# Autodesk Inventor assembly: ASY Beshkino main
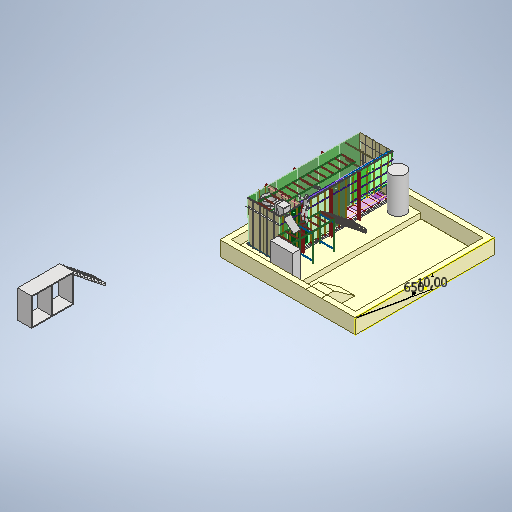
[picture p0: Inventor's stored thumbnail of the model, 512x512]
Saved by Autodesk Inventor 2025 (Build 290162010, 162A)
## iProperties
Created: 2024-08-27
Part Number: ASY Beshkino main
Document SubType Name: Assembly
Designer: DELL
Author: DELL
## Documents named in this file (13)
- C:\Users\DELL\YandexDisk-badmisterfox\домашниий пк\Inventor\BSH_Beshkino_bio_tank\ASY Beshkino main.iam
- C:\Users\DELL\YandexDisk-badmisterfox\домашниий пк\Inventor\BSH_Beshkino_bio_tank\BSH 0 foudation.ipt
- C:\Users\DELL\YandexDisk-badmisterfox\домашниий пк\Inventor\BSH_Beshkino_bio_tank\ASY Beshkino_bio_tank.iam
- C:\Users\DELL\YandexDisk-badmisterfox\домашниий пк\Inventor\BSH_Beshkino_bio_tank\ASY Trommel.iam
- C:\Users\DELL\YandexDisk-badmisterfox\домашниий пк\Inventor\BSH_Beshkino_bio_tank\3d party\RXm3 assieme dimensionale mag2018.ipt
- C:\Users\DELL\YandexDisk-badmisterfox\домашниий пк\Inventor\BSH_Beshkino_bio_tank\3d party\motor-reductor NMRV040\motor-reductor NMRV040.iam
- C:\Users\DELL\YandexDisk-badmisterfox\домашниий пк\Inventor\BSH_Beshkino_bio_tank\BSH 01 foam filter.ipt
- C:\Users\DELL\YandexDisk-badmisterfox\домашниий пк\Inventor\BSH_Beshkino_bio_tank\BSH 01 bag.ipt
- C:\Users\DELL\YandexDisk-badmisterfox\домашниий пк\Inventor\BSH_Beshkino_bio_tank\BSH 03 upstairs.ipt
- C:\Users\DELL\YandexDisk-badmisterfox\домашниий пк\Inventor\BSH_Beshkino_bio_tank\Конструкция.iam
- C:\Users\DELL\YandexDisk-badmisterfox\домашниий пк\Inventor\BSH_Beshkino_bio_tank\лестница\Перегородка\ASY NDM 11.030 перегородка рама 2 горизонт.iam
- C:\Users\DELL\YandexDisk-badmisterfox\домашниий пк\Inventor\BSH_Beshkino_bio_tank\ISO 657_15 - SB 140x15 - 3000.ipt
- C:\Users\DELL\YandexDisk-badmisterfox\домашниий пк\Inventor\BSH_Beshkino_bio_tank\лестница\dummi\human 01\ч ASY human dummy 01.iam
## Components (19 placed, 12 different names)
1. BSH 0 foudation:1 — Mate:1, Mate:2, Mate:3, Mate:4, Flush:2, Flush:3, Flush:4, Mate:7
2. ASY Beshkino_bio_tank:1 [sub-assembly] — Mate:2, Mate:3, Mate:4, Flush:1, Mate:5, Mate:6, Mate:8, Mate:10, Flush:7, Mate:14
3. ASY Trommel:1 [sub-assembly] — Flush:1
4. RXm3 assieme dimensionale mag2018:1 — Mate:5
5. RXm3 assieme dimensionale mag2018:2 — Mate:6
6. motor-reductor NMRV040:1 [sub-assembly]
7. BSH 01 foam filter:1 — Flush:2
8. BSH 01 bag:1 — Flush:3
9. BSH 03 upstairs:1 — Flush:4
10. Конструкция:1 [sub-assembly] — Mate:7, Mate:8, Mate:13
11. ASY NDM 11.030 перегородка рама 2 горизонт:1 [sub-assembly] — Flush:5, Flush:6, Mate:9, Mate:10
12. ASY NDM 11.030 перегородка рама 2 горизонт:2 [sub-assembly] — Flush:5, Flush:6, Mate:9
13. ч ASY human dummy 01:1 [sub-assembly] — Mate:13
14. ISO 657_15 - SB 140x15 - 3000:1 — Flush:7, Mate:14
15. ISO 657_15 - SB 140x15 - 3000:2
16. ISO 657_15 - SB 140x15 - 3000:3
17. ISO 657_15 - SB 140x15 - 3000:4
18. ISO 657_15 - SB 140x15 - 3000:5
19. ISO 657_15 - SB 140x15 - 3000:6
## Component patterns: (6 elements, first: ISO 657_15 - SB 140x15 - 3000:1)
## Relationships (19: Mate 12, Flush 7)
- Mate:1: BSH 0 foudation:1
- Mate:2: BSH 0 foudation:1 ↔ ASY Beshkino_bio_tank:1
- Mate:3 (100 mm): BSH 0 foudation:1 ↔ ASY Beshkino_bio_tank:1
- Mate:4 (200 mm): BSH 0 foudation:1 ↔ ASY Beshkino_bio_tank:1
- Flush:1: ASY Beshkino_bio_tank:1 ↔ ASY Trommel:1
- Mate:5: ASY Beshkino_bio_tank:1 ↔ RXm3 assieme dimensionale mag2018:1
- Mate:6: ASY Beshkino_bio_tank:1 ↔ RXm3 assieme dimensionale mag2018:2
- Flush:2: BSH 0 foudation:1 ↔ BSH 01 foam filter:1
- Flush:3: BSH 0 foudation:1 ↔ BSH 01 bag:1
- Flush:4: BSH 0 foudation:1 ↔ BSH 03 upstairs:1
- Mate:7: BSH 0 foudation:1 ↔ Конструкция:1
- Mate:8 (140 mm): ASY Beshkino_bio_tank:1 ↔ Конструкция:1
- Flush:5: ASY NDM 11.030 перегородка рама 2 горизонт:1 ↔ ASY NDM 11.030 перегородка рама 2 горизонт:2
- Flush:6: ASY NDM 11.030 перегородка рама 2 горизонт:1 ↔ ASY NDM 11.030 перегородка рама 2 горизонт:2
- Mate:9: ASY NDM 11.030 перегородка рама 2 горизонт:1 ↔ ASY NDM 11.030 перегородка рама 2 горизонт:2
- Mate:10: ASY Beshkino_bio_tank:1 ↔ ASY NDM 11.030 перегородка рама 2 горизонт:1
- Mate:13: Конструкция:1 ↔ ч ASY human dummy 01:1
- Flush:7 (1500 mm): ASY Beshkino_bio_tank:1 ↔ ISO 657_15 - SB 140x15 - 3000:1
- Mate:14: ASY Beshkino_bio_tank:1 ↔ ISO 657_15 - SB 140x15 - 3000:1
